# Autodesk Inventor assembly: WheelIntake4.0
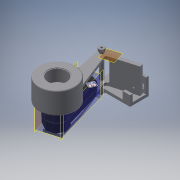
[picture p0: Inventor's stored thumbnail of the model, 180x180]
Saved by Autodesk Inventor 2017 (Build 210142000, 142)
## iProperties
Created: 2017-12-13
Part Number: WheelIntake4.0
Document SubType Name: Assembly
Designer: User
Author: User
## Documents named in this file (6)
- C:\Robotics\CAD\2017-18_CAD\WheelIntake4.0.iam
- C:\Robotics\CAD\COTSParts\Rev\REV-41-1300.ipt
- C:\Robotics\CAD\2017-18_CAD\WheelIntakeMount4.0.ipt
- C:\Robotics\CAD\COTSParts\Fasteners\97345A171_TYPE 316 STAINLESS STEEL SHOULDER SCREW.ipt
- C:\Robotics\CAD\2017-18_CAD\WheelIntake4.0Base.ipt
- C:\Robotics\CAD\COTSParts\Wheels\2.5inFoamWheel250TMD.ipt
## Components (5 placed, 5 different names)
1. REV-41-1300:1 — Insert:1, Insert:2
2. WheelIntakeMount4.0:1 — Insert:1, Insert:2, Insert:3, Insert:5
3. 97345A171_TYPE 316 STAINLESS STEEL SHOULDER SCREW:1 — Insert:3, Insert:4
4. WheelIntake4.0Base:1 — Insert:4, Mate:1
5. 2.5inFoamWheel250TMD:1 — Insert:5, Mate:1
## Relationships (6: Insert 5, Mate 1)
- Insert:1: REV-41-1300:1 ↔ WheelIntakeMount4.0:1
- Insert:2: REV-41-1300:1 ↔ WheelIntakeMount4.0:1
- Insert:3 (3.175 mm): WheelIntakeMount4.0:1 ↔ 97345A171_TYPE 316 STAINLESS STEEL SHOULDER SCREW:1
- Insert:4: 97345A171_TYPE 316 STAINLESS STEEL SHOULDER SCREW:1 ↔ WheelIntake4.0Base:1
- Insert:5: WheelIntakeMount4.0:1 ↔ 2.5inFoamWheel250TMD:1
- Mate:1 (-25.4 mm): WheelIntake4.0Base:1 ↔ 2.5inFoamWheel250TMD:1
